# Autodesk Inventor assembly: Assembly_Cube_SQUID_Z_Focus_v3
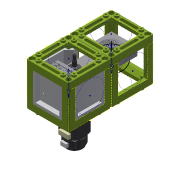
[picture p0: Inventor's stored thumbnail of the model, 180x180]
Saved by Autodesk Inventor 2022 (Build 260153000, 153)
## iProperties
Created: 2020-11-11
Part Number: Assembly_Cube_SQUID_Z_Focus_v3
Document SubType Name: Assembly
Designer: marsikovabarbora
Author: marsikovabarbora
## Documents named in this file (7)
- C:\Users\PrakashLab\Documents\UC2-INVENTOR-Git\uc2_v3\Assembly_Cube_SQUID_Z_Focus_v3.iam
- C:\Users\PrakashLab\Documents\UC2-INVENTOR-Git\uc2_v3\Assembly_Cube_empty_IM_v3.iam
- C:\Users\PrakashLab\Documents\UC2-INVENTOR-Git\uc2_v3\00_X-axis_MX25-SC.iam
- C:\Users\PrakashLab\Documents\UC2-INVENTOR-Git\uc2_v3\SQUID\AMETEK-21H4U-2_5-0_75-12-ENC.ipt
- C:\Users\PrakashLab\Documents\UC2-INVENTOR-Git\uc2_v3\30_Cube_SQUID_Z_Focus_base_v3.ipt
- C:\Users\PrakashLab\Documents\UC2-INVENTOR-Git\uc2_v3\30_Cube_SQUID_Z_Focus_slide_v3.ipt
- C:\Users\PrakashLab\Documents\UC2-INVENTOR-Git\uc2_v3\30_Cube_SQUID_Z_Focus_spacer_v3.ipt
## Components (7 placed, 6 different names)
1. 30_Cube_SQUID_Z_Focus_base_v3:1 — Mate:10, Mate:11, Mate:12, Mate:19, Mate:20, Mate:21, Flush:1, Flush:2
2. 00_X-axis_MX25-SC:1 [sub-assembly] — Mate:19, Mate:20, Mate:21, Insert:1
3. 30_Cube_SQUID_Z_Focus_slide_v3:1 — Insert:1, Angle:1
4. 30_Cube_SQUID_Z_Focus_spacer_v3:1 — Flush:1, Flush:2, Insert:2
5. AMETEK-21H4U-2_5-0_75-12-ENC:1 — Insert:2
6. Assembly_Cube_empty_IM_v3:1 [sub-assembly] — Mate:1, Mate:2, Mate:3, Mate:10, Mate:11, Mate:12
7. Assembly_Cube_empty_IM_v3:2 [sub-assembly] — Angle:1
## Component patterns: (2 elements, first: Assembly_Cube_empty_IM_v3:1)
## Relationships (14: Mate 9, Insert 2, Flush 2, Angle 1)
- Mate:1: Assembly_Cube_empty_IM_v3:1
- Mate:2: Assembly_Cube_empty_IM_v3:1
- Mate:3: Assembly_Cube_empty_IM_v3:1
- Mate:10: 30_Cube_SQUID_Z_Focus_base_v3:1 ↔ Assembly_Cube_empty_IM_v3:1
- Mate:11: 30_Cube_SQUID_Z_Focus_base_v3:1 ↔ Assembly_Cube_empty_IM_v3:1
- Mate:12: 30_Cube_SQUID_Z_Focus_base_v3:1 ↔ Assembly_Cube_empty_IM_v3:1
- Mate:19: 30_Cube_SQUID_Z_Focus_base_v3:1 ↔ 00_X-axis_MX25-SC:1
- Mate:20: 30_Cube_SQUID_Z_Focus_base_v3:1 ↔ 00_X-axis_MX25-SC:1
- Mate:21 (-5 mm): 30_Cube_SQUID_Z_Focus_base_v3:1 ↔ 00_X-axis_MX25-SC:1
- Insert:1: 00_X-axis_MX25-SC:1 ↔ 30_Cube_SQUID_Z_Focus_slide_v3:1
- Angle:1 (0 deg): 30_Cube_SQUID_Z_Focus_slide_v3:1 ↔ Assembly_Cube_empty_IM_v3:2
- Flush:1: 30_Cube_SQUID_Z_Focus_base_v3:1 ↔ 30_Cube_SQUID_Z_Focus_spacer_v3:1
- Flush:2: 30_Cube_SQUID_Z_Focus_base_v3:1 ↔ 30_Cube_SQUID_Z_Focus_spacer_v3:1
- Insert:2: 30_Cube_SQUID_Z_Focus_spacer_v3:1 ↔ AMETEK-21H4U-2_5-0_75-12-ENC:1
